# Autodesk Inventor assembly: roller complete
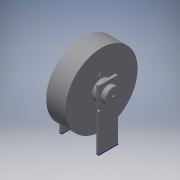
[picture p0: Inventor's stored thumbnail of the model, 180x180]
Saved by Autodesk Inventor 2019 (Build 230136000, 136)
## iProperties
Created: 2020-02-15
Part Number: roller complete
Document SubType Name: Assembly
Designer: Admin
Author: Admin
## Documents named in this file (4)
- C:\Users\Admin\Documents\Exploration\roller complete.iam
- C:\Users\Admin\Documents\Exploration\roller.ipt
- C:\Users\Admin\Documents\Exploration\roller pin.ipt
- C:\Users\Admin\Documents\Exploration\roller support.ipt
## Components (4 placed, 3 different names)
1. roller:2 — Rigid:1
2. roller pin:1 — Rigid:1, Rotational:1, Rigid:2
3. roller support:1 — Rotational:1
4. roller support:2 — Rigid:2
## Relationships (3: WeldJoint 2, RevoluteJoint 1)
- Rigid:1 [WeldJoint] (15 mm): roller:2 ↔ roller pin:1
- Rotational:1 [RevoluteJoint]: roller pin:1 ↔ roller support:1
- Rigid:2 [WeldJoint]: roller pin:1 ↔ roller support:2
